# Autodesk Inventor assembly: LINK3
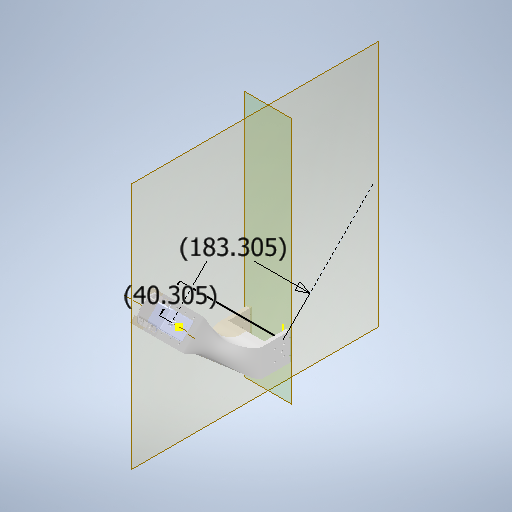
[picture p0: Inventor's stored thumbnail of the model, 512x512]
Saved by Autodesk Inventor 2026.1 (Build 301233020, 233B)
## iProperties
Created: 2025-10-15
Part Number: LINK3
Document SubType Name: Assembly
Designer: wlgns
Author: wlgns
## Documents named in this file (3)
- C:\Users\wlgns\Desktop\project\ARA Project\ARA_CAD_model\ARA_v2\LINK3.iam
- C:\Users\wlgns\Desktop\project\ARA Project\ARA_CAD_model\ARA_v2\ARM_2 SKETCH - smooth.ipt
- C:\Users\wlgns\Desktop\project\ARA Project\ARA_CAD_model\ARA_v2\MX-28T_MIR.ipt
## Components (2 placed, 2 different names)
1. ARM_2 SKETCH - smooth:1 — 메이트:1, 메이트:2, 메이트:3, 메이트:4, 메이트:5, 메이트:9, 각도:1, 플러쉬:1
2. MX-28T_MIR:1 — 메이트:7, 메이트:8, 메이트:9, 각도:1
## Relationships (10: Mate 8, Angle 1, Flush 1)
- 메이트:1 [Mate] (-17.7 mm): ARM_2 SKETCH - smooth:1
- 메이트:2 [Mate] (-3 mm): ARM_2 SKETCH - smooth:1
- 메이트:3 [Mate]: ARM_2 SKETCH - smooth:1
- 메이트:4 [Mate]: ARM_2 SKETCH - smooth:1
- 메이트:5 [Mate]: ARM_2 SKETCH - smooth:1
- 메이트:7 [Mate]: MX-28T_MIR:1
- 메이트:8 [Mate]: MX-28T_MIR:1
- 메이트:9 [Mate]: ARM_2 SKETCH - smooth:1 ↔ MX-28T_MIR:1
- 각도:1 [Angle] (180 deg): ARM_2 SKETCH - smooth:1 ↔ MX-28T_MIR:1
- 플러쉬:1 [Flush] (-3 mm): ARM_2 SKETCH - smooth:1
